# Autodesk Inventor assembly: caterpillar_module_final_B
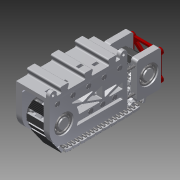
[picture p0: Inventor's stored thumbnail of the model, 180x180]
Saved by Autodesk Inventor 2015 (Build 190159000, 159)
## iProperties
Created: 2016-07-10
Part Number: caterpillar_module_final_B
Document SubType Name: Assembly
Designer: JavierPC
Author: JavierPC
## Documents named in this file (17)
- D:\Mis Documentos\TFM\CAD\v2\assembly\caterpillar_module_final_B.iam
- D:\Mis Documentos\TFM\CAD\v2\parts\combined_base_caterpillar_narrow_A_21.ipt
- D:\Mis Documentos\TFM\CAD\v2\parts\support_caterpillar_lateral_v31.ipt
- C:\Users\JavierPC\Documents\Inventor\Content Center Files\R2015\es-ES\DIN BEARING(1)\DIN 625 SKF - SKF 618_8.ipt
- D:\Mis Documentos\TFM\CAD\v2\parts\sprocket_encoder_axis_left_21.ipt
- D:\Mis Documentos\TFM\CAD\v2\parts\dumper_base_v1_SOCKET1.ipt
- D:\Mis Documentos\TFM\CAD\v2\parts\spring_axis1.ipt
- D:\Mis Documentos\TFM\CAD\v2\parts\support_caterpillar_spring_v1.31.ipt
- D:\Mis Documentos\TFM\CAD\v2\parts\sprocket_back_axis_21.ipt
- D:\Mis Documentos\TFM\CAD\v2\parts\Alignment_narrow1.ipt
- D:\Mis Documentos\TFM\CAD\v2\parts\spring_final1.iam
- C:\Users\JavierPC\Documents\Inventor\Content Center Files\R2015\es-ES\ISO 4032(1)\ISO 4032 - M2DIN EN.ipt
- C:\Users\JavierPC\Documents\Inventor\Content Center Files\R2015\es-ES\ISO 2009(1)\ISO 2009 - M2 x 12DIN EN 10.ipt
- D:\Mis Documentos\TFM\CAD\v2\parts\dumper_v9_NS1.ipt
- D:\Mis Documentos\TFM\CAD\v2\parts\chain_path1.ipt
- D:\Mis Documentos\TFM\CAD\v2\parts\chain_shoe35.iam
- D:\Mis Documentos\TFM\CAD\v2\parts\link_joint_v4_z15_Dr1.51.ipt
## Components (112 placed, 16 different names)
1. combined_base_caterpillar_narrow_A_21:1 — Coincidencia:3, Coincidencia:2, Coincidencia:1, Coincidencia:6, Coincidencia:5, Coincidencia:4, Nivelación:1, Coincidencia:7, Coincidencia:11, Insertar:5, Insertar:6, Coincidencia:22, Coincidencia:26, Ángulo:4, Insertar:12, Ángulo:5, Insertar:13, Ángulo:3, Insertar:11, Ángulo:2, Insertar:10, Ángulo:1, Insertar:9, Insertar:28, Insertar:29, Insertar:30
2. support_caterpillar_lateral_v31:1 — Coincidencia:6, Coincidencia:5, Coincidencia:4, Nivelación:2, Coincidencia:8, Insertar:2, Insertar:1, Insertar:3, Insertar:4, Nivelación:102, Coincidencia:105, Coincidencia:24, Insertar:20, Insertar:21, Insertar:22, Insertar:23, Insertar:24, Insertar:25, Insertar:26, Insertar:27
3. DIN 625 SKF 618/8:1 — Nivelación:3, Coincidencia:16, Coincidencia:20
4. DIN 625 SKF 618/8:2 — Nivelación:4, Coincidencia:17, Coincidencia:19, Coincidencia:18
5. DIN 625 SKF 618/8:3 — Nivelación:2, Coincidencia:8
6. DIN 625 SKF 618/8:4 — Nivelación:1, Coincidencia:7, Coincidencia:10, Coincidencia:9
7. sprocket_encoder_axis_left_21:1 — Coincidencia:10, Coincidencia:9, planoCentral
8. dumper_base_v1_SOCKET1:1 — Insertar:2, Insertar:1, Coincidencia:11, Ángulo:9, Insertar:17, Ángulo:10, Insertar:18, Ángulo:8, Insertar:16, Ángulo:11, Insertar:19, Ángulo:7, Insertar:15, Ángulo:6, Insertar:14, Nivelación:6, Coincidencia:34, Coincidencia:33
9. spring_axis1:1 — Insertar:3, Coincidencia:14, Insertar:7
10. spring_axis1:2 — Insertar:4, Coincidencia:15, Insertar:8, Coincidencia:25
11. spring_axis1:3 — Insertar:5, Coincidencia:13, Coincidencia:27
12. spring_axis1:4 — Insertar:6, Coincidencia:12, Coincidencia:23
13. support_caterpillar_spring_v1.31:1 — Nivelación:3, Coincidencia:16, Coincidencia:15, Coincidencia:14, Coincidencia:29, Coincidencia:30
14. support_caterpillar_spring_v1.31:2 — Nivelación:4, Coincidencia:17, Coincidencia:13, Coincidencia:12, Coincidencia:31, Coincidencia:32
15. sprocket_back_axis_21:1 — Coincidencia:20, Coincidencia:19, Coincidencia:18
16. Alignment_narrow1:1 — Insertar:8, Insertar:7
17. spring_final1:1 [sub-assembly] — Nivelación:102, Coincidencia:105, Coincidencia:29
18. spring_final1:2 [sub-assembly] — Coincidencia:31, Coincidencia:23, Coincidencia:22
19. spring_final1:3 [sub-assembly] — Coincidencia:30, Coincidencia:25, Coincidencia:24
20. spring_final1:4 [sub-assembly] — Coincidencia:32, Coincidencia:27, Coincidencia:26
21. DIN EN 24032 M2:1 — Ángulo:9, Insertar:17
22. DIN EN 24032 M2:2 — Ángulo:10, Insertar:18
23. DIN EN 24032 M2:3 — Ángulo:8, Insertar:16
24. DIN EN 24032 M2:4 — Ángulo:4, Insertar:12
25. DIN EN 24032 M2:5 — Ángulo:5, Insertar:13
26. DIN EN 24032 M2:6 — Ángulo:11, Insertar:19
27. DIN EN 24032 M2:7 — Ángulo:7, Insertar:15
28. DIN EN 24032 M2:8 — Ángulo:6, Insertar:14
29. DIN EN 24032 M2:9 — Ángulo:3, Insertar:11
30. DIN EN 24032 M2:10 — Ángulo:2, Insertar:10
31. DIN EN 24032 M2:11 — Ángulo:1, Insertar:9
32. DIN EN ISO 2009 M2 x 12:1 — Insertar:20
33. DIN EN ISO 2009 M2 x 12:2 — Insertar:21
34. DIN EN ISO 2009 M2 x 12:3 — Insertar:22
35. DIN EN ISO 2009 M2 x 12:4 — Insertar:23
36. DIN EN ISO 2009 M2 x 12:5 — Insertar:24
37. DIN EN ISO 2009 M2 x 12:6 — Insertar:25
38. DIN EN ISO 2009 M2 x 12:7 — Insertar:26
39. DIN EN ISO 2009 M2 x 12:8 — Insertar:27
40. DIN EN ISO 2009 M2 x 12:9 — Insertar:28
41. DIN EN ISO 2009 M2 x 12:10 — Insertar:29
42. DIN EN ISO 2009 M2 x 12:11 — Insertar:30
43. dumper_v9_NS1:1 — Nivelación:6, Coincidencia:34, Coincidencia:33
44. chain_path1:1 — planoCentral, Nivelación:37, Coincidencia:37, Nivelación:38, Coincidencia:39, Nivelación:39, Nivelación:41, Nivelación:40, Nivelación:42, Nivelación:43, Nivelación:44, Nivelación:45, Nivelación:46, Nivelación:47, Nivelación:48, Nivelación:49, Nivelación:50, Nivelación:51, Nivelación:53, Nivelación:55, Nivelación:57, Nivelación:59, Nivelación:58, Nivelación:54, Nivelación:56, Nivelación:52, Nivelación:60, Nivelación:61, Nivelación:62, Nivelación:63, Nivelación:64, Nivelación:65, Nivelación:66, Nivelación:67, Nivelación:68, Nivelación:69, Nivelación:70, Nivelación:71, Nivelación:72, Nivelación:73, Nivelación:74, Nivelación:75, Nivelación:76, Nivelación:77, Nivelación:78, Nivelación:79, Nivelación:80, Nivelación:81, Nivelación:82, Nivelación:83, Nivelación:84, Nivelación:85, Nivelación:97, Nivelación:96, Nivelación:95, Nivelación:94, Nivelación:93, Nivelación:92, Nivelación:91, Nivelación:90, Nivelación:89, Nivelación:88, Nivelación:87, Nivelación:86, Nivelación:98, Nivelación:99, Nivelación:100, Nivelación:101, Nivelación:103
45. chain_shoe35:1 [sub-assembly] — Nivelación:37, Coincidencia:36, Coincidencia:99
46. link_joint_v4_z15_Dr1.51:1 — Coincidencia:37, Coincidencia:36, Coincidencia:40
47. chain_shoe35:2 [sub-assembly] — Coincidencia:40, Nivelación:38, Coincidencia:38
48. link_joint_v4_z15_Dr1.51:2 — Coincidencia:39, Coincidencia:38, Coincidencia:44
49. chain_shoe35:3 [sub-assembly] — Coincidencia:44, Nivelación:39, Coincidencia:41
50. link_joint_v4_z15_Dr1.51:3 — Nivelación:41, Coincidencia:41, Coincidencia:43
51. chain_shoe35:4 [sub-assembly] — Nivelación:40, Coincidencia:43, Coincidencia:42
52. link_joint_v4_z15_Dr1.51:4 — Nivelación:42, Coincidencia:42, Coincidencia:52
53. chain_shoe35:5 [sub-assembly] — Coincidencia:52, Nivelación:43, Coincidencia:45
54. link_joint_v4_z15_Dr1.51:5 — Nivelación:44, Coincidencia:45, Coincidencia:47
55. chain_shoe35:6 [sub-assembly] — Nivelación:45, Coincidencia:47, Coincidencia:46
56. link_joint_v4_z15_Dr1.51:6 — Nivelación:46, Coincidencia:46, Coincidencia:51
57. chain_shoe35:7 [sub-assembly] — Nivelación:47, Coincidencia:51, Coincidencia:48
58. link_joint_v4_z15_Dr1.51:7 — Nivelación:48, Coincidencia:48, Coincidencia:50
59. chain_shoe35:8 [sub-assembly] — Nivelación:49, Coincidencia:50, Coincidencia:49
60. link_joint_v4_z15_Dr1.51:8 — Nivelación:50, Coincidencia:49, Coincidencia:53
61. chain_shoe35:9 [sub-assembly] — Coincidencia:53, Nivelación:51, Coincidencia:54
62. chain_shoe35:10 [sub-assembly] — Nivelación:53, Coincidencia:56, Coincidencia:55
63. chain_shoe35:11 [sub-assembly] — Nivelación:55, Coincidencia:57, Coincidencia:58
64. chain_shoe35:12 [sub-assembly] — Nivelación:57, Coincidencia:60, Coincidencia:59
65. chain_shoe35:13 [sub-assembly] — Nivelación:59, Coincidencia:61, Coincidencia:87
66. link_joint_v4_z15_Dr1.51:9 — Coincidencia:61, Nivelación:58, Coincidencia:60
67. link_joint_v4_z15_Dr1.51:10 — Coincidencia:57, Nivelación:54, Coincidencia:56
68. link_joint_v4_z15_Dr1.51:11 — Coincidencia:59, Nivelación:56, Coincidencia:58
69. link_joint_v4_z15_Dr1.51:12 — Coincidencia:55, Nivelación:52, Coincidencia:54
70. chain_shoe35:14 [sub-assembly] — Nivelación:60, Coincidencia:62, Coincidencia:86
71. link_joint_v4_z15_Dr1.51:13 — Nivelación:61, Coincidencia:62, Coincidencia:64
72. chain_shoe35:15 [sub-assembly] — Nivelación:62, Coincidencia:64, Coincidencia:63
73. link_joint_v4_z15_Dr1.51:14 — Nivelación:63, Coincidencia:63, Coincidencia:68
74. chain_shoe35:16 [sub-assembly] — Nivelación:64, Coincidencia:68, Coincidencia:65
75. link_joint_v4_z15_Dr1.51:15 — Nivelación:65, Coincidencia:65, Coincidencia:67
76. chain_shoe35:17 [sub-assembly] — Nivelación:66, Coincidencia:67, Coincidencia:66
77. link_joint_v4_z15_Dr1.51:16 — Nivelación:67, Coincidencia:66, Coincidencia:76
78. chain_shoe35:18 [sub-assembly] — Nivelación:68, Coincidencia:76, Coincidencia:69
79. link_joint_v4_z15_Dr1.51:17 — Nivelación:69, Coincidencia:69, Coincidencia:71
80. chain_shoe35:19 [sub-assembly] — Nivelación:70, Coincidencia:71, Coincidencia:70
81. link_joint_v4_z15_Dr1.51:18 — Nivelación:71, Coincidencia:70, Coincidencia:75
82. chain_shoe35:20 [sub-assembly] — Nivelación:72, Coincidencia:75, Coincidencia:72
83. link_joint_v4_z15_Dr1.51:19 — Nivelación:73, Coincidencia:72, Coincidencia:74
84. chain_shoe35:21 [sub-assembly] — Nivelación:74, Coincidencia:74, Coincidencia:73
85. link_joint_v4_z15_Dr1.51:20 — Nivelación:75, Coincidencia:73, Coincidencia:77
86. chain_shoe35:22 [sub-assembly] — Nivelación:76, Coincidencia:77, Coincidencia:78
87. chain_shoe35:23 [sub-assembly] — Nivelación:77, Coincidencia:80, Coincidencia:79
88. chain_shoe35:24 [sub-assembly] — Nivelación:78, Coincidencia:81, Coincidencia:82
89. chain_shoe35:25 [sub-assembly] — Nivelación:79, Coincidencia:84, Coincidencia:83
90. chain_shoe35:26 [sub-assembly] — Nivelación:80, Coincidencia:85, Coincidencia:107
91. link_joint_v4_z15_Dr1.51:21 — Nivelación:81, Coincidencia:85, Coincidencia:84
92. link_joint_v4_z15_Dr1.51:22 — Nivelación:82, Coincidencia:80, Coincidencia:81
93. link_joint_v4_z15_Dr1.51:23 — Nivelación:83, Coincidencia:83, Coincidencia:82
94. link_joint_v4_z15_Dr1.51:24 — Nivelación:84, Coincidencia:79, Coincidencia:78
95. link_joint_v4_z15_Dr1.51:25 — Coincidencia:87, Coincidencia:86, Nivelación:85
96. chain_shoe35:27 [sub-assembly] — Nivelación:97, Coincidencia:88, Coincidencia:103
97. link_joint_v4_z15_Dr1.51:26 — Nivelación:96, Coincidencia:88, Coincidencia:90
98. chain_shoe35:28 [sub-assembly] — Nivelación:95, Coincidencia:90, Coincidencia:89
99. link_joint_v4_z15_Dr1.51:27 — Nivelación:94, Coincidencia:89, Coincidencia:94
100. chain_shoe35:29 [sub-assembly] — Nivelación:93, Coincidencia:94, Coincidencia:91
101. link_joint_v4_z15_Dr1.51:28 — Nivelación:92, Coincidencia:91, Coincidencia:93
102. chain_shoe35:30 [sub-assembly] — Nivelación:91, Coincidencia:93, Coincidencia:92
103. link_joint_v4_z15_Dr1.51:29 — Nivelación:90, Coincidencia:92, Coincidencia:98
104. chain_shoe35:31 [sub-assembly] — Nivelación:89, Coincidencia:98, Coincidencia:95
105. link_joint_v4_z15_Dr1.51:30 — Nivelación:88, Coincidencia:95, Coincidencia:97
106. chain_shoe35:32 [sub-assembly] — Nivelación:87, Coincidencia:97, Coincidencia:96
107. link_joint_v4_z15_Dr1.51:31 — Coincidencia:99, Nivelación:86, Coincidencia:96
108. chain_shoe35:33 [sub-assembly] — Nivelación:98, Coincidencia:100, Coincidencia:106
109. link_joint_v4_z15_Dr1.51:32 — Nivelación:99, Coincidencia:100, Coincidencia:102
110. chain_shoe35:34 [sub-assembly] — Nivelación:100, Coincidencia:102, Coincidencia:104
111. link_joint_v4_z15_Dr1.51:33 — Coincidencia:104, Coincidencia:103, Nivelación:101
112. link_joint_v4_z15_Dr1.51:34 — Coincidencia:107, Coincidencia:106, Nivelación:103
## Relationships (217: Mate 168, Insert 30, Angle 11, Flush 8)
- Coincidencia:3 [Mate]: combined_base_caterpillar_narrow_A_21:1
- Coincidencia:2 [Flush]: combined_base_caterpillar_narrow_A_21:1
- Coincidencia:1 [Mate]: combined_base_caterpillar_narrow_A_21:1
- Coincidencia:6 [Mate]: combined_base_caterpillar_narrow_A_21:1 ↔ support_caterpillar_lateral_v31:1
- Coincidencia:5 [Mate]: combined_base_caterpillar_narrow_A_21:1 ↔ support_caterpillar_lateral_v31:1
- Coincidencia:4 [Mate]: combined_base_caterpillar_narrow_A_21:1 ↔ support_caterpillar_lateral_v31:1
- Nivelación:2 [Flush]: support_caterpillar_lateral_v31:1 ↔ DIN 625 SKF 618/8:3
- Coincidencia:8 [Mate]: support_caterpillar_lateral_v31:1 ↔ DIN 625 SKF 618/8:3
- Nivelación:1 [Flush]: combined_base_caterpillar_narrow_A_21:1 ↔ DIN 625 SKF 618/8:4
- Coincidencia:7 [Mate]: combined_base_caterpillar_narrow_A_21:1 ↔ DIN 625 SKF 618/8:4
- Coincidencia:10 [Mate]: DIN 625 SKF 618/8:4 ↔ sprocket_encoder_axis_left_21:1
- Coincidencia:9 [Mate]: DIN 625 SKF 618/8:4 ↔ sprocket_encoder_axis_left_21:1
- Insertar:2: support_caterpillar_lateral_v31:1 ↔ dumper_base_v1_SOCKET1:1
- Insertar:1: support_caterpillar_lateral_v31:1 ↔ dumper_base_v1_SOCKET1:1
- Coincidencia:11 [Mate]: combined_base_caterpillar_narrow_A_21:1 ↔ dumper_base_v1_SOCKET1:1
- Insertar:3: support_caterpillar_lateral_v31:1 ↔ spring_axis1:1
- Insertar:4: support_caterpillar_lateral_v31:1 ↔ spring_axis1:2
- Insertar:5: combined_base_caterpillar_narrow_A_21:1 ↔ spring_axis1:3
- Insertar:6: combined_base_caterpillar_narrow_A_21:1 ↔ spring_axis1:4
- Nivelación:3 [Flush]: DIN 625 SKF 618/8:1 ↔ support_caterpillar_spring_v1.31:1
- Coincidencia:16 [Mate]: DIN 625 SKF 618/8:1 ↔ support_caterpillar_spring_v1.31:1
- Coincidencia:15 [Mate]: spring_axis1:2 ↔ support_caterpillar_spring_v1.31:1
- Coincidencia:14 [Mate]: spring_axis1:1 ↔ support_caterpillar_spring_v1.31:1
- Nivelación:4 [Flush]: DIN 625 SKF 618/8:2 ↔ support_caterpillar_spring_v1.31:2
- Coincidencia:17 [Mate]: DIN 625 SKF 618/8:2 ↔ support_caterpillar_spring_v1.31:2
- Coincidencia:13 [Mate]: spring_axis1:3 ↔ support_caterpillar_spring_v1.31:2
- Coincidencia:12 [Mate]: spring_axis1:4 ↔ support_caterpillar_spring_v1.31:2
- Coincidencia:20 [Mate]: DIN 625 SKF 618/8:1 ↔ sprocket_back_axis_21:1
- Coincidencia:19 [Mate]: DIN 625 SKF 618/8:2 ↔ sprocket_back_axis_21:1
- Coincidencia:18 [Mate]: DIN 625 SKF 618/8:2 ↔ sprocket_back_axis_21:1
- Insertar:8: spring_axis1:2 ↔ Alignment_narrow1:1
- Insertar:7: spring_axis1:1 ↔ Alignment_narrow1:1
- Nivelación:102 [Mate]: support_caterpillar_lateral_v31:1 ↔ spring_final1:1
- Coincidencia:105 [Mate]: support_caterpillar_lateral_v31:1 ↔ spring_final1:1
- Coincidencia:29 [Mate]: support_caterpillar_spring_v1.31:1 ↔ spring_final1:1
- Coincidencia:31 [Mate]: support_caterpillar_spring_v1.31:2 ↔ spring_final1:2
- Coincidencia:23 [Mate]: spring_axis1:4 ↔ spring_final1:2
- Coincidencia:22 [Mate]: combined_base_caterpillar_narrow_A_21:1 ↔ spring_final1:2
- Coincidencia:30 [Mate]: support_caterpillar_spring_v1.31:1 ↔ spring_final1:3
- Coincidencia:25 [Mate]: spring_axis1:2 ↔ spring_final1:3
- Coincidencia:24 [Mate]: support_caterpillar_lateral_v31:1 ↔ spring_final1:3
- Coincidencia:32 [Mate]: support_caterpillar_spring_v1.31:2 ↔ spring_final1:4
- Coincidencia:27 [Mate]: spring_axis1:3 ↔ spring_final1:4
- Coincidencia:26 [Mate]: combined_base_caterpillar_narrow_A_21:1 ↔ spring_final1:4
- Ángulo:9 [Angle] (0 deg): dumper_base_v1_SOCKET1:1 ↔ DIN EN 24032 M2:1
- Insertar:17: dumper_base_v1_SOCKET1:1 ↔ DIN EN 24032 M2:1
- Ángulo:10 [Angle] (0 deg): dumper_base_v1_SOCKET1:1 ↔ DIN EN 24032 M2:2
- Insertar:18: dumper_base_v1_SOCKET1:1 ↔ DIN EN 24032 M2:2
- Ángulo:8 [Angle] (0 deg): dumper_base_v1_SOCKET1:1 ↔ DIN EN 24032 M2:3
- Insertar:16: dumper_base_v1_SOCKET1:1 ↔ DIN EN 24032 M2:3
- Ángulo:4 [Angle] (0 deg): combined_base_caterpillar_narrow_A_21:1 ↔ DIN EN 24032 M2:4
- Insertar:12: combined_base_caterpillar_narrow_A_21:1 ↔ DIN EN 24032 M2:4
- Ángulo:5 [Angle] (0 deg): combined_base_caterpillar_narrow_A_21:1 ↔ DIN EN 24032 M2:5
- Insertar:13: combined_base_caterpillar_narrow_A_21:1 ↔ DIN EN 24032 M2:5
- Ángulo:11 [Angle] (0 deg): dumper_base_v1_SOCKET1:1 ↔ DIN EN 24032 M2:6
- Insertar:19: dumper_base_v1_SOCKET1:1 ↔ DIN EN 24032 M2:6
- Ángulo:7 [Angle] (0 deg): dumper_base_v1_SOCKET1:1 ↔ DIN EN 24032 M2:7
- Insertar:15: dumper_base_v1_SOCKET1:1 ↔ DIN EN 24032 M2:7
- Ángulo:6 [Angle] (0 deg): dumper_base_v1_SOCKET1:1 ↔ DIN EN 24032 M2:8
- Insertar:14: dumper_base_v1_SOCKET1:1 ↔ DIN EN 24032 M2:8
- Ángulo:3 [Angle] (0 deg): combined_base_caterpillar_narrow_A_21:1 ↔ DIN EN 24032 M2:9
- Insertar:11: combined_base_caterpillar_narrow_A_21:1 ↔ DIN EN 24032 M2:9
- Ángulo:2 [Angle] (0 deg): combined_base_caterpillar_narrow_A_21:1 ↔ DIN EN 24032 M2:10
- Insertar:10: combined_base_caterpillar_narrow_A_21:1 ↔ DIN EN 24032 M2:10
- Ángulo:1 [Angle] (0 deg): combined_base_caterpillar_narrow_A_21:1 ↔ DIN EN 24032 M2:11
- Insertar:9: combined_base_caterpillar_narrow_A_21:1 ↔ DIN EN 24032 M2:11
- Insertar:20: support_caterpillar_lateral_v31:1 ↔ DIN EN ISO 2009 M2 x 12:1
- Insertar:21: support_caterpillar_lateral_v31:1 ↔ DIN EN ISO 2009 M2 x 12:2
- Insertar:22: support_caterpillar_lateral_v31:1 ↔ DIN EN ISO 2009 M2 x 12:3
- Insertar:23: support_caterpillar_lateral_v31:1 ↔ DIN EN ISO 2009 M2 x 12:4
- Insertar:24: support_caterpillar_lateral_v31:1 ↔ DIN EN ISO 2009 M2 x 12:5
- Insertar:25: support_caterpillar_lateral_v31:1 ↔ DIN EN ISO 2009 M2 x 12:6
- Insertar:26: support_caterpillar_lateral_v31:1 ↔ DIN EN ISO 2009 M2 x 12:7
- Insertar:27: support_caterpillar_lateral_v31:1 ↔ DIN EN ISO 2009 M2 x 12:8
- Insertar:28: combined_base_caterpillar_narrow_A_21:1 ↔ DIN EN ISO 2009 M2 x 12:9
- Insertar:29: combined_base_caterpillar_narrow_A_21:1 ↔ DIN EN ISO 2009 M2 x 12:10
- Insertar:30: combined_base_caterpillar_narrow_A_21:1 ↔ DIN EN ISO 2009 M2 x 12:11
- Nivelación:6 [Flush]: dumper_base_v1_SOCKET1:1 ↔ dumper_v9_NS1:1
- Coincidencia:34 [Mate]: dumper_base_v1_SOCKET1:1 ↔ dumper_v9_NS1:1
- Coincidencia:33 [Mate]: dumper_base_v1_SOCKET1:1 ↔ dumper_v9_NS1:1
- planoCentral [Mate]: sprocket_encoder_axis_left_21:1 ↔ chain_path1:1
- Nivelación:37 [Mate]: chain_path1:1 ↔ chain_shoe35:1
- Coincidencia:37 [Flush]: chain_path1:1 ↔ link_joint_v4_z15_Dr1.51:1
- Coincidencia:36 [Mate]: chain_shoe35:1 ↔ link_joint_v4_z15_Dr1.51:1
- Coincidencia:40 [Mate]: link_joint_v4_z15_Dr1.51:1 ↔ chain_shoe35:2
- Nivelación:38 [Mate]: chain_path1:1 ↔ chain_shoe35:2
- Coincidencia:39 [Flush]: chain_path1:1 ↔ link_joint_v4_z15_Dr1.51:2
- Coincidencia:38 [Mate]: chain_shoe35:2 ↔ link_joint_v4_z15_Dr1.51:2
- Coincidencia:44 [Mate]: link_joint_v4_z15_Dr1.51:2 ↔ chain_shoe35:3
- Nivelación:39 [Mate]: chain_path1:1 ↔ chain_shoe35:3
- Nivelación:41 [Mate]: chain_path1:1 ↔ link_joint_v4_z15_Dr1.51:3
- Coincidencia:41 [Mate]: chain_shoe35:3 ↔ link_joint_v4_z15_Dr1.51:3
- Nivelación:40 [Mate]: chain_path1:1 ↔ chain_shoe35:4
- Coincidencia:43 [Mate]: link_joint_v4_z15_Dr1.51:3 ↔ chain_shoe35:4
- Nivelación:42 [Mate]: chain_path1:1 ↔ link_joint_v4_z15_Dr1.51:4
- Coincidencia:42 [Mate]: chain_shoe35:4 ↔ link_joint_v4_z15_Dr1.51:4
- Coincidencia:52 [Mate]: link_joint_v4_z15_Dr1.51:4 ↔ chain_shoe35:5
- Nivelación:43 [Mate]: chain_path1:1 ↔ chain_shoe35:5
- Nivelación:44 [Mate]: chain_path1:1 ↔ link_joint_v4_z15_Dr1.51:5
- Coincidencia:45 [Mate]: chain_shoe35:5 ↔ link_joint_v4_z15_Dr1.51:5
- Nivelación:45 [Mate]: chain_path1:1 ↔ chain_shoe35:6
- Coincidencia:47 [Mate]: link_joint_v4_z15_Dr1.51:5 ↔ chain_shoe35:6
- Nivelación:46 [Mate]: chain_path1:1 ↔ link_joint_v4_z15_Dr1.51:6
- Coincidencia:46 [Mate]: chain_shoe35:6 ↔ link_joint_v4_z15_Dr1.51:6
- Nivelación:47 [Mate]: chain_path1:1 ↔ chain_shoe35:7
- Coincidencia:51 [Mate]: link_joint_v4_z15_Dr1.51:6 ↔ chain_shoe35:7
- Nivelación:48 [Mate]: chain_path1:1 ↔ link_joint_v4_z15_Dr1.51:7
- Coincidencia:48 [Mate]: chain_shoe35:7 ↔ link_joint_v4_z15_Dr1.51:7
- Nivelación:49 [Mate]: chain_path1:1 ↔ chain_shoe35:8
- Coincidencia:50 [Mate]: link_joint_v4_z15_Dr1.51:7 ↔ chain_shoe35:8
- Nivelación:50 [Mate]: chain_path1:1 ↔ link_joint_v4_z15_Dr1.51:8
- Coincidencia:49 [Mate]: chain_shoe35:8 ↔ link_joint_v4_z15_Dr1.51:8
- Coincidencia:53 [Mate]: link_joint_v4_z15_Dr1.51:8 ↔ chain_shoe35:9
- Nivelación:51 [Mate]: chain_path1:1 ↔ chain_shoe35:9
- Nivelación:53 [Mate]: chain_path1:1 ↔ chain_shoe35:10
- Nivelación:55 [Mate]: chain_path1:1 ↔ chain_shoe35:11
- Nivelación:57 [Mate]: chain_path1:1 ↔ chain_shoe35:12
- Nivelación:59 [Mate]: chain_path1:1 ↔ chain_shoe35:13
- Coincidencia:61 [Mate]: chain_shoe35:13 ↔ link_joint_v4_z15_Dr1.51:9
- Nivelación:58 [Mate]: chain_path1:1 ↔ link_joint_v4_z15_Dr1.51:9
- Coincidencia:60 [Mate]: chain_shoe35:12 ↔ link_joint_v4_z15_Dr1.51:9
- Coincidencia:57 [Mate]: chain_shoe35:11 ↔ link_joint_v4_z15_Dr1.51:10
- Nivelación:54 [Mate]: chain_path1:1 ↔ link_joint_v4_z15_Dr1.51:10
- Coincidencia:56 [Mate]: chain_shoe35:10 ↔ link_joint_v4_z15_Dr1.51:10
- Coincidencia:59 [Mate]: chain_shoe35:12 ↔ link_joint_v4_z15_Dr1.51:11
- Nivelación:56 [Mate]: chain_path1:1 ↔ link_joint_v4_z15_Dr1.51:11
- Coincidencia:58 [Mate]: chain_shoe35:11 ↔ link_joint_v4_z15_Dr1.51:11
- Coincidencia:55 [Mate]: chain_shoe35:10 ↔ link_joint_v4_z15_Dr1.51:12
- Nivelación:52 [Mate]: chain_path1:1 ↔ link_joint_v4_z15_Dr1.51:12
- Coincidencia:54 [Mate]: chain_shoe35:9 ↔ link_joint_v4_z15_Dr1.51:12
- Nivelación:60 [Mate]: chain_path1:1 ↔ chain_shoe35:14
- Nivelación:61 [Mate]: chain_path1:1 ↔ link_joint_v4_z15_Dr1.51:13
- Coincidencia:62 [Mate]: chain_shoe35:14 ↔ link_joint_v4_z15_Dr1.51:13
- Nivelación:62 [Mate]: chain_path1:1 ↔ chain_shoe35:15
- Coincidencia:64 [Mate]: link_joint_v4_z15_Dr1.51:13 ↔ chain_shoe35:15
- Nivelación:63 [Mate]: chain_path1:1 ↔ link_joint_v4_z15_Dr1.51:14
- Coincidencia:63 [Mate]: chain_shoe35:15 ↔ link_joint_v4_z15_Dr1.51:14
- Nivelación:64 [Mate]: chain_path1:1 ↔ chain_shoe35:16
- Coincidencia:68 [Mate]: link_joint_v4_z15_Dr1.51:14 ↔ chain_shoe35:16
- Nivelación:65 [Mate]: chain_path1:1 ↔ link_joint_v4_z15_Dr1.51:15
- Coincidencia:65 [Mate]: chain_shoe35:16 ↔ link_joint_v4_z15_Dr1.51:15
- Nivelación:66 [Mate]: chain_path1:1 ↔ chain_shoe35:17
- Coincidencia:67 [Mate]: link_joint_v4_z15_Dr1.51:15 ↔ chain_shoe35:17
- Nivelación:67 [Mate]: chain_path1:1 ↔ link_joint_v4_z15_Dr1.51:16
- Coincidencia:66 [Mate]: chain_shoe35:17 ↔ link_joint_v4_z15_Dr1.51:16
- Nivelación:68 [Mate]: chain_path1:1 ↔ chain_shoe35:18
- Coincidencia:76 [Mate]: link_joint_v4_z15_Dr1.51:16 ↔ chain_shoe35:18
- Nivelación:69 [Mate]: chain_path1:1 ↔ link_joint_v4_z15_Dr1.51:17
- Coincidencia:69 [Mate]: chain_shoe35:18 ↔ link_joint_v4_z15_Dr1.51:17
- Nivelación:70 [Mate]: chain_path1:1 ↔ chain_shoe35:19
- Coincidencia:71 [Mate]: link_joint_v4_z15_Dr1.51:17 ↔ chain_shoe35:19
- Nivelación:71 [Mate]: chain_path1:1 ↔ link_joint_v4_z15_Dr1.51:18
- Coincidencia:70 [Mate]: chain_shoe35:19 ↔ link_joint_v4_z15_Dr1.51:18
- Nivelación:72 [Mate]: chain_path1:1 ↔ chain_shoe35:20
- Coincidencia:75 [Mate]: link_joint_v4_z15_Dr1.51:18 ↔ chain_shoe35:20
- Nivelación:73 [Mate]: chain_path1:1 ↔ link_joint_v4_z15_Dr1.51:19
- Coincidencia:72 [Mate]: chain_shoe35:20 ↔ link_joint_v4_z15_Dr1.51:19
- Nivelación:74 [Mate]: chain_path1:1 ↔ chain_shoe35:21
- Coincidencia:74 [Mate]: link_joint_v4_z15_Dr1.51:19 ↔ chain_shoe35:21
- Nivelación:75 [Mate]: chain_path1:1 ↔ link_joint_v4_z15_Dr1.51:20
- Coincidencia:73 [Mate]: chain_shoe35:21 ↔ link_joint_v4_z15_Dr1.51:20
- Nivelación:76 [Mate]: chain_path1:1 ↔ chain_shoe35:22
- Coincidencia:77 [Mate]: link_joint_v4_z15_Dr1.51:20 ↔ chain_shoe35:22
- Nivelación:77 [Mate]: chain_path1:1 ↔ chain_shoe35:23
- Nivelación:78 [Mate]: chain_path1:1 ↔ chain_shoe35:24
- Nivelación:79 [Mate]: chain_path1:1 ↔ chain_shoe35:25
- Nivelación:80 [Mate]: chain_path1:1 ↔ chain_shoe35:26
- Nivelación:81 [Mate]: chain_path1:1 ↔ link_joint_v4_z15_Dr1.51:21
- Coincidencia:85 [Mate]: chain_shoe35:26 ↔ link_joint_v4_z15_Dr1.51:21
- Coincidencia:84 [Mate]: chain_shoe35:25 ↔ link_joint_v4_z15_Dr1.51:21
- Nivelación:82 [Mate]: chain_path1:1 ↔ link_joint_v4_z15_Dr1.51:22
- Coincidencia:80 [Mate]: chain_shoe35:23 ↔ link_joint_v4_z15_Dr1.51:22
- Coincidencia:81 [Mate]: chain_shoe35:24 ↔ link_joint_v4_z15_Dr1.51:22
- Nivelación:83 [Mate]: chain_path1:1 ↔ link_joint_v4_z15_Dr1.51:23
- Coincidencia:83 [Mate]: chain_shoe35:25 ↔ link_joint_v4_z15_Dr1.51:23
- Coincidencia:82 [Mate]: chain_shoe35:24 ↔ link_joint_v4_z15_Dr1.51:23
- Nivelación:84 [Mate]: chain_path1:1 ↔ link_joint_v4_z15_Dr1.51:24
- Coincidencia:79 [Mate]: chain_shoe35:23 ↔ link_joint_v4_z15_Dr1.51:24
- Coincidencia:78 [Mate]: chain_shoe35:22 ↔ link_joint_v4_z15_Dr1.51:24
- Coincidencia:87 [Mate]: chain_shoe35:13 ↔ link_joint_v4_z15_Dr1.51:25
- Coincidencia:86 [Mate]: chain_shoe35:14 ↔ link_joint_v4_z15_Dr1.51:25
- Nivelación:85 [Mate]: chain_path1:1 ↔ link_joint_v4_z15_Dr1.51:25
- Nivelación:97 [Mate]: chain_path1:1 ↔ chain_shoe35:27
- Nivelación:96 [Mate]: chain_path1:1 ↔ link_joint_v4_z15_Dr1.51:26
- Coincidencia:88 [Mate]: chain_shoe35:27 ↔ link_joint_v4_z15_Dr1.51:26
- Nivelación:95 [Mate]: chain_path1:1 ↔ chain_shoe35:28
- Coincidencia:90 [Mate]: link_joint_v4_z15_Dr1.51:26 ↔ chain_shoe35:28
- Nivelación:94 [Mate]: chain_path1:1 ↔ link_joint_v4_z15_Dr1.51:27
- Coincidencia:89 [Mate]: chain_shoe35:28 ↔ link_joint_v4_z15_Dr1.51:27
- Nivelación:93 [Mate]: chain_path1:1 ↔ chain_shoe35:29
- Coincidencia:94 [Mate]: link_joint_v4_z15_Dr1.51:27 ↔ chain_shoe35:29
- Nivelación:92 [Mate]: chain_path1:1 ↔ link_joint_v4_z15_Dr1.51:28
- Coincidencia:91 [Mate]: chain_shoe35:29 ↔ link_joint_v4_z15_Dr1.51:28
- Nivelación:91 [Mate]: chain_path1:1 ↔ chain_shoe35:30
- Coincidencia:93 [Mate]: link_joint_v4_z15_Dr1.51:28 ↔ chain_shoe35:30
- Nivelación:90 [Mate]: chain_path1:1 ↔ link_joint_v4_z15_Dr1.51:29
- Coincidencia:92 [Mate]: chain_shoe35:30 ↔ link_joint_v4_z15_Dr1.51:29
- Nivelación:89 [Mate]: chain_path1:1 ↔ chain_shoe35:31
- Coincidencia:98 [Mate]: link_joint_v4_z15_Dr1.51:29 ↔ chain_shoe35:31
- Nivelación:88 [Mate]: chain_path1:1 ↔ link_joint_v4_z15_Dr1.51:30
- Coincidencia:95 [Mate]: chain_shoe35:31 ↔ link_joint_v4_z15_Dr1.51:30
- Nivelación:87 [Mate]: chain_path1:1 ↔ chain_shoe35:32
- Coincidencia:97 [Mate]: link_joint_v4_z15_Dr1.51:30 ↔ chain_shoe35:32
- Coincidencia:99 [Mate]: chain_shoe35:1 ↔ link_joint_v4_z15_Dr1.51:31
- Nivelación:86 [Mate]: chain_path1:1 ↔ link_joint_v4_z15_Dr1.51:31
- Coincidencia:96 [Mate]: chain_shoe35:32 ↔ link_joint_v4_z15_Dr1.51:31
- Nivelación:98 [Mate]: chain_path1:1 ↔ chain_shoe35:33
- Nivelación:99 [Mate]: chain_path1:1 ↔ link_joint_v4_z15_Dr1.51:32
- Coincidencia:100 [Mate]: chain_shoe35:33 ↔ link_joint_v4_z15_Dr1.51:32
- Nivelación:100 [Mate]: chain_path1:1 ↔ chain_shoe35:34
- Coincidencia:102 [Mate]: link_joint_v4_z15_Dr1.51:32 ↔ chain_shoe35:34
- Coincidencia:104 [Mate]: chain_shoe35:34 ↔ link_joint_v4_z15_Dr1.51:33
- Coincidencia:103 [Mate]: chain_shoe35:27 ↔ link_joint_v4_z15_Dr1.51:33
- Nivelación:101 [Mate]: chain_path1:1 ↔ link_joint_v4_z15_Dr1.51:33
- Coincidencia:107 [Mate]: chain_shoe35:26 ↔ link_joint_v4_z15_Dr1.51:34
- Coincidencia:106 [Mate]: chain_shoe35:33 ↔ link_joint_v4_z15_Dr1.51:34
- Nivelación:103 [Mate]: chain_path1:1 ↔ link_joint_v4_z15_Dr1.51:34
